# Autodesk Inventor assembly: gear_box
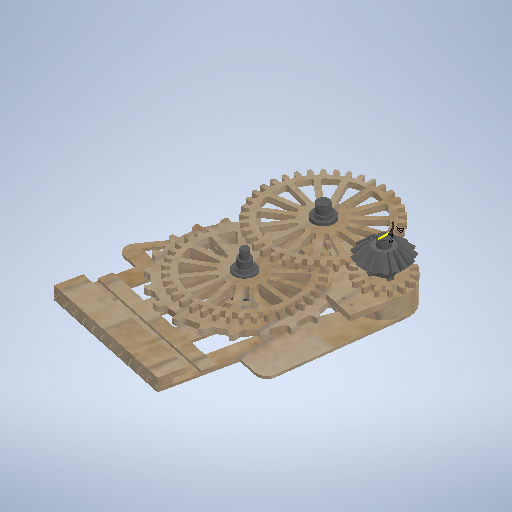
[picture p0: Inventor's stored thumbnail of the model, 512x512]
Saved by Autodesk Inventor 2026.1 (Build 301233020, 233B)
## iProperties
Created: 2025-09-25
Part Number: gear_box
Document SubType Name: Assembly
Designer: hibik
Author: hibik
## Documents named in this file (11)
- C:\Users\hibik\Documents\Robomech\conveyer\power_module\gear_box.iam
- C:\Users\hibik\Documents\Robomech\conveyer\power_module\gear_box_base.iam
- C:\Users\hibik\Documents\Robomech\conveyer\power_module\M3_38.ipt
- C:\Users\hibik\Documents\Robomech\conveyer\power_module\roller.ipt
- C:\Users\hibik\Documents\Robomech\conveyer\power_module\spacer.ipt
- C:\Users\hibik\Documents\Robomech\conveyer\power_module\axis_middle.ipt
- C:\Users\hibik\Documents\Robomech\conveyer\power_module\M3_15.ipt
- C:\Users\hibik\Documents\Robomech\conveyer\power_module\axis_out.ipt
- C:\Users\hibik\Documents\Robomech\conveyer\power_module\axis_in.ipt
- C:\Users\hibik\Documents\Robomech\conveyer\power_module\M3_15_input.ipt
- C:\Users\hibik\Documents\Robomech\conveyer\power_module\M3_15_crown_out.ipt
## Components (11 placed, 10 different names)
1. gear_box_base:1 [sub-assembly] — 挿入:2, 挿入:4, 角度:1, 挿入:6, 挿入:7, 挿入:8
2. M3_38:1 — 挿入:1, フラッシュ:1
3. roller:1 — 挿入:1, フラッシュ:1, 挿入:3
4. spacer:1 — 挿入:2, 挿入:3
5. axis_middle:1 — 挿入:4, 角度:1
6. M3_15:1 — 挿入:5, 挿入:7
7. M3_38:2 — 挿入:5
8. axis_out:1 — 挿入:6
9. axis_in:1 — 挿入:8, 挿入:12
10. M3_15_input:1 — 挿入:12, メイト:3, メイト:4, メイト:5
11. M3_15_crown_out:1 — メイト:3, メイト:4, メイト:5
## Relationships (14: Insert 9, Mate 3, Flush 1, Angle 1)
- 挿入:1 [Insert]: M3_38:1 ↔ roller:1
- フラッシュ:1 [Flush]: M3_38:1 ↔ roller:1
- 挿入:2 [Insert]: gear_box_base:1 ↔ spacer:1
- 挿入:3 [Insert]: roller:1 ↔ spacer:1
- 挿入:4 [Insert]: gear_box_base:1 ↔ axis_middle:1
- 角度:1 [Angle] (180 deg): gear_box_base:1 ↔ axis_middle:1
- 挿入:5 [Insert]: M3_15:1 ↔ M3_38:2
- 挿入:6 [Insert]: gear_box_base:1 ↔ axis_out:1
- 挿入:7 [Insert] (0.5 mm): gear_box_base:1 ↔ M3_15:1
- 挿入:8 [Insert]: gear_box_base:1 ↔ axis_in:1
- 挿入:12 [Insert]: axis_in:1 ↔ M3_15_input:1
- メイト:3 [Mate]: M3_15_input:1 ↔ M3_15_crown_out:1
- メイト:4 [Mate]: M3_15_input:1 ↔ M3_15_crown_out:1
- メイト:5 [Mate]: M3_15_input:1 ↔ M3_15_crown_out:1
